# Autodesk Inventor assembly: WormAndMotorizedRingFor3dPrintingV02
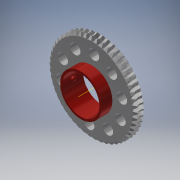
[picture p0: Inventor's stored thumbnail of the model, 180x180]
Saved by Autodesk Inventor 2019.3 (Build 233278000, 278)
## iProperties
Created: 2019-01-29
Part Number: WormAndMotorizedRingFor3dPrintingV02
Document SubType Name: Assembly
Designer: steele
Author: steele
## Documents named in this file (3)
- C:\git\CAD-Development\robSteele\ShapeWays\TelescopeProjects\Focuser\WormAndMotorizedRingFor3dPrintingV02.iam
- C:\git\CAD-Development\robSteele\ShapeWays\TelescopeProjects\Focuser\WormDrive02\Design Accelerator\Worm Gear1.ipt
- C:\git\CAD-Development\robSteele\ShapeWays\TelescopeProjects\Focuser\ExternalMotorizedOuterRing.ipt
## Components (2 placed, 2 different names)
1. Worm Gear:1 — Insert:1
2. ExternalMotorizedOuterRing:1 — Insert:1
## Relationships (1: Insert 1)
- Insert:1: Worm Gear:1 ↔ ExternalMotorizedOuterRing:1
